# Autodesk Inventor assembly: Robot-Game-Piece-Funnel
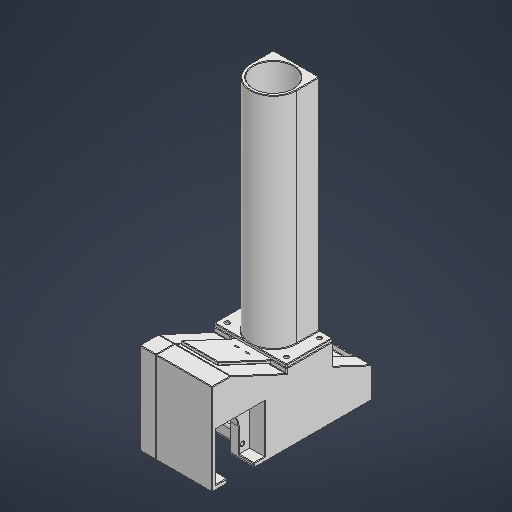
[picture p0: Inventor's stored thumbnail of the model, 512x512]
Saved by Autodesk Inventor 2025 (Build 290162010, 162A)
## iProperties
Created: 2025-12-03
Part Number: Robot-Game-Piece-Funnel
Document SubType Name: Assembly
Designer: FizzyApple12
Author: FizzyApple12
## Documents named in this file (6)
- C:\Users\FizzyApple12\Desktop\connect-4-robot\mcad\Robot-Game-Piece-Funnel\Robot-Game-Piece-Funnel.iam
- C:\Users\FizzyApple12\Desktop\connect-4-robot\mcad\Robot-Game-Piece-Funnel\Game-Piece-Funnel-Motor-Half.ipt
- C:\Users\FizzyApple12\Desktop\connect-4-robot\mcad\Robot-Game-Piece-Funnel\Game-Piece-Funnel-Enclosure-Half.ipt
- C:\Users\FizzyApple12\Desktop\connect-4-robot\mcad\Robot-Game-Piece-Funnel\Game-Piece-Funnel-Hopper.ipt
- C:\Users\FizzyApple12\Desktop\connect-4-robot\mcad\Robot-Game-Piece-Funnel\Game-Piece-Funnel-Pusher-Plate.ipt
- C:\Users\FizzyApple12\Desktop\connect-4-robot\mcad\Robot-Game-Piece-Funnel\Game-Piece-Funnel-Pusher-Carriage.ipt
## Components (5 placed, 5 different names)
1. Game-Piece-Funnel-Motor-Half:1
2. Game-Piece-Funnel-Enclosure-Half:1
3. Game-Piece-Funnel-Hopper:1
4. Game-Piece-Funnel-Pusher-Plate:1
5. Game-Piece-Funnel-Pusher-Carriage:1
## Relationships (11: Mate 11)
- [Mate]: Game-Piece-Funnel-Motor-Half:1 ↔ Game-Piece-Funnel-Enclosure-Half:1
- [Mate]: Game-Piece-Funnel-Motor-Half:1 ↔ Game-Piece-Funnel-Enclosure-Half:1
- [Mate]: Game-Piece-Funnel-Motor-Half:1 ↔ Game-Piece-Funnel-Enclosure-Half:1
- [Mate]: Game-Piece-Funnel-Motor-Half:1 ↔ Game-Piece-Funnel-Hopper:1
- [Mate]: Game-Piece-Funnel-Motor-Half:1 ↔ Game-Piece-Funnel-Hopper:1
- [Mate]: Game-Piece-Funnel-Enclosure-Half:1 ↔ Game-Piece-Funnel-Hopper:1
- [Mate]: Game-Piece-Funnel-Motor-Half:1 ↔ Game-Piece-Funnel-Pusher-Plate:1
- [Mate] (1 mm): Game-Piece-Funnel-Motor-Half:1 ↔ Game-Piece-Funnel-Pusher-Plate:1
- [Mate]: Game-Piece-Funnel-Pusher-Plate:1 ↔ Game-Piece-Funnel-Pusher-Carriage:1
- [Mate]: Game-Piece-Funnel-Pusher-Plate:1 ↔ Game-Piece-Funnel-Pusher-Carriage:1
- [Mate]: Game-Piece-Funnel-Pusher-Plate:1 ↔ Game-Piece-Funnel-Pusher-Carriage:1
